# Autodesk Inventor assembly: head_long_side
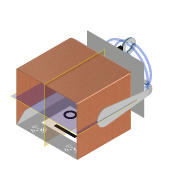
[picture p0: Inventor's stored thumbnail of the model, 180x180]
Saved by Autodesk Inventor 2021.1 (Build 251245010, 245A)
## iProperties
Created: 2023-01-27
Part Number: head_long_side
Document SubType Name: Assembly
Designer: zmoze
Author: zmoze
## Documents named in this file (16)
- C:\Users\zmoze\OneDrive\Рабочий стол\GrabCAD\Smile_2022-2023\олимпиада\head_long_side.iam
- C:\Users\zmoze\OneDrive\Рабочий стол\GrabCAD\Smile_2022-2023\олимпиада\face_long_side.ipt
- C:\Users\zmoze\OneDrive\Рабочий стол\GrabCAD\Smile_2022-2023\олимпиада\head_without_face_long_side.ipt
- C:\Users\zmoze\OneDrive\Рабочий стол\GrabCAD\Smile_2022-2023\олимпиада\head_mind_long_side.iam
- C:\Users\zmoze\OneDrive\Рабочий стол\GrabCAD\Smile_2022-2023\олимпиада\electronic_plate_long_side.ipt
- C:\Users\zmoze\OneDrive\Рабочий стол\GrabCAD\Smile_2022-2023\олимпиада\arduino_MEGA2560.iam
- C:\Users\zmoze\OneDrive\Рабочий стол\GrabCAD\Smile_2022-2023\олимпиада\рот.ipt
- C:\Users\zmoze\OneDrive\Рабочий стол\GrabCAD\Smile_2022-2023\олимпиада\глаз.ipt
- C:\Users\zmoze\OneDrive\Рабочий стол\GrabCAD\Smile_2022-2023\олимпиада\mini_servo.ipt
- C:\Users\zmoze\OneDrive\Рабочий стол\GrabCAD\Smile_2022-2023\олимпиада\ухо.ipt
- C:\Users\zmoze\OneDrive\Рабочий стол\GrabCAD\Smile_2022-2023\олимпиада\mount_on_servo.ipt
- C:\Users\zmoze\OneDrive\Рабочий стол\GrabCAD\Smile_2022-2023\олимпиада\Motor_Driver.ipt
- C:\Users\zmoze\OneDrive\Рабочий стол\GrabCAD\Smile_2022-2023\олимпиада\gyro.iam
- C:\Users\zmoze\OneDrive\Рабочий стол\GrabCAD\Smile_2022-2023\олимпиада\аккум.ipt
- C:\Users\zmoze\OneDrive\Рабочий стол\GrabCAD\Smile_2022-2023\олимпиада\стабилизатор.ipt
- C:\Users\zmoze\OneDrive\Рабочий стол\GrabCAD\Smile_2022-2023\олимпиада\крепление_аккума.ipt
## Components (20 placed, 15 different names)
1. head_without_face_long_side:1 — Совмещение:1, Совмещение:2, Заподлицо:1, Совмещение:3, Совмещение:4, Заподлицо:2, Совмещение:5, Совмещение:6, Заподлицо:3, Совмещение:13, Совмещение:14, Совмещение:15, Заподлицо:7, Заподлицо:8, Заподлицо:9, Угол:1, Угол:2, Угол:3, Угол:4, Совмещение:29, Заподлицо:10, Совмещение:30
2. face_long_side:1 — Совмещение:1, Совмещение:2, Заподлицо:1, Заподлицо:4, Заподлицо:5, Заподлицо:6, Совмещение:7, Совмещение:8, Совмещение:9, Совмещение:10, Совмещение:11, Совмещение:12
3. electronic_plate_long_side:1 — Совмещение:5, Совмещение:6, Заподлицо:3, Совмещение:24, Совмещение:25, Совмещение:26, Совмещение:27, Совмещение:28, Совмещение:31, Совмещение:32
4. head_mind_long_side:1 [sub-assembly] — Совмещение:3, Совмещение:4, Заподлицо:2
5. arduino_MEGA2560:1 [sub-assembly] — Совмещение:25
6. рот:1 — Заподлицо:6, Совмещение:7, Совмещение:8
7. глаз:1 — Заподлицо:5, Совмещение:10, Совмещение:12
8. глаз:2 — Заподлицо:4, Совмещение:9, Совмещение:11
9. mini_servo:1 — Совмещение:13, Заподлицо:8, Заподлицо:9, Совмещение:18, Совмещение:19
10. mini_servo:2 — Совмещение:14, Совмещение:15, Заподлицо:7, Совмещение:16, Совмещение:17
11. mount_on_servo:1 — Совмещение:18, Совмещение:19, Совмещение:22, Совмещение:23, Угол:3
12. mount_on_servo:2 — Совмещение:16, Совмещение:17, Совмещение:20, Совмещение:21, Угол:4
13. ухо:1 — Совмещение:22, Совмещение:23, Угол:2
14. ухо:2 — Совмещение:20, Совмещение:21, Угол:1
15. Motor_Driver:1 — Совмещение:24
16. gyro:1 [sub-assembly] — Совмещение:26
17. аккум:1 — Совмещение:27, Совмещение:29, Заподлицо:10, Совмещение:33, Совмещение:34, Заподлицо:11, Заподлицо:12
18. стабилизатор:1 — Совмещение:28, Совмещение:30
19. крепление_аккума:1 — Совмещение:32, Совмещение:33, Заподлицо:12
20. крепление_аккума:2 — Совмещение:31, Совмещение:34, Заподлицо:11
## Relationships (50: Mate 34, Flush 12, Angle 4)
- Совмещение:1 [Mate]: head_without_face_long_side:1 ↔ face_long_side:1
- Совмещение:2 [Mate]: head_without_face_long_side:1 ↔ face_long_side:1
- Заподлицо:1 [Flush]: head_without_face_long_side:1 ↔ face_long_side:1
- Совмещение:3 [Mate] (70 mm): head_without_face_long_side:1 ↔ head_mind_long_side:1
- Совмещение:4 [Mate]: head_without_face_long_side:1 ↔ head_mind_long_side:1
- Заподлицо:2 [Flush]: head_without_face_long_side:1 ↔ head_mind_long_side:1
- Совмещение:5 [Mate]: head_without_face_long_side:1 ↔ electronic_plate_long_side:1
- Совмещение:6 [Mate]: head_without_face_long_side:1 ↔ electronic_plate_long_side:1
- Заподлицо:3 [Flush]: head_without_face_long_side:1 ↔ electronic_plate_long_side:1
- Заподлицо:4 [Flush]: face_long_side:1 ↔ глаз:2
- Заподлицо:5 [Flush]: face_long_side:1 ↔ глаз:1
- Заподлицо:6 [Flush]: face_long_side:1 ↔ рот:1
- Совмещение:7 [Mate] (20 mm): face_long_side:1 ↔ рот:1
- Совмещение:8 [Mate] (47.75 mm): face_long_side:1 ↔ рот:1
- Совмещение:9 [Mate] (40 mm): face_long_side:1 ↔ глаз:2
- Совмещение:10 [Mate] (40 mm): face_long_side:1 ↔ глаз:1
- Совмещение:11 [Mate] (40 mm): face_long_side:1 ↔ глаз:2
- Совмещение:12 [Mate] (40 mm): face_long_side:1 ↔ глаз:1
- Совмещение:13 [Mate]: head_without_face_long_side:1 ↔ mini_servo:1
- Совмещение:14 [Mate]: head_without_face_long_side:1 ↔ mini_servo:2
- Совмещение:15 [Mate]: head_without_face_long_side:1 ↔ mini_servo:2
- Заподлицо:7 [Flush]: head_without_face_long_side:1 ↔ mini_servo:2
- Заподлицо:8 [Flush]: head_without_face_long_side:1 ↔ mini_servo:1
- Заподлицо:9 [Flush]: head_without_face_long_side:1 ↔ mini_servo:1
- Совмещение:16 [Mate]: mini_servo:2 ↔ mount_on_servo:2
- Совмещение:17 [Mate]: mini_servo:2 ↔ mount_on_servo:2
- Совмещение:18 [Mate]: mini_servo:1 ↔ mount_on_servo:1
- Совмещение:19 [Mate]: mini_servo:1 ↔ mount_on_servo:1
- Совмещение:20 [Mate]: mount_on_servo:2 ↔ ухо:2
- Совмещение:21 [Mate]: mount_on_servo:2 ↔ ухо:2
- Совмещение:22 [Mate]: mount_on_servo:1 ↔ ухо:1
- Совмещение:23 [Mate]: mount_on_servo:1 ↔ ухо:1
- Угол:1 [Angle] (0 deg): head_without_face_long_side:1 ↔ ухо:2
- Угол:2 [Angle] (180 deg): head_without_face_long_side:1 ↔ ухо:1
- Угол:3 [Angle] (0 deg): head_without_face_long_side:1 ↔ mount_on_servo:1
- Угол:4 [Angle] (0 deg): head_without_face_long_side:1 ↔ mount_on_servo:2
- Совмещение:24 [Mate] (20 mm): electronic_plate_long_side:1 ↔ Motor_Driver:1
- Совмещение:25 [Mate] (20 mm): electronic_plate_long_side:1 ↔ arduino_MEGA2560:1
- Совмещение:26 [Mate] (20 mm): electronic_plate_long_side:1 ↔ gyro:1
- Совмещение:27 [Mate]: electronic_plate_long_side:1 ↔ аккум:1
- Совмещение:28 [Mate]: electronic_plate_long_side:1 ↔ стабилизатор:1
- Совмещение:29 [Mate]: head_without_face_long_side:1 ↔ аккум:1
- Заподлицо:10 [Flush] (50 mm): head_without_face_long_side:1 ↔ аккум:1
- Совмещение:30 [Mate]: head_without_face_long_side:1 ↔ стабилизатор:1
- Совмещение:31 [Mate]: electronic_plate_long_side:1 ↔ крепление_аккума:2
- Совмещение:32 [Mate]: electronic_plate_long_side:1 ↔ крепление_аккума:1
- Совмещение:33 [Mate]: аккум:1 ↔ крепление_аккума:1
- Совмещение:34 [Mate]: аккум:1 ↔ крепление_аккума:2
- Заподлицо:11 [Flush] (-20 mm): аккум:1 ↔ крепление_аккума:2
- Заподлицо:12 [Flush] (-20 mm): аккум:1 ↔ крепление_аккума:1
